# Autodesk Inventor assembly: 0070.725-R
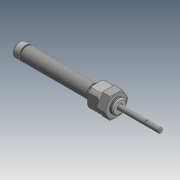
[picture p0: Inventor's stored thumbnail of the model, 180x180]
Saved by Autodesk Inventor 2020.4 (Build 244396000, 396)
## iProperties
Part Number: 0070.725-R
Catalog Web Link: www.cadenas.de
Description: Original Line Standard Air Cylinders-Standard Air Cylinders
Vendor: BIMBA
Document SubType Name: Assembly
Designer: partserver
Manufacturer: BIMBA
Mass: 4.93332 g
Surface Area: 61.3507 cm^2
Volume: 4.93332 cm^3
Density: 1 g/cm^3
Category: PARTsolutions
Company: BIMBA
PSOL_IDENT_0: {$CADENAS_DATA\23d-libs\bimba\bimba_brand\bimba_imperial\bimba_full_line\original_line_cylinders\sta
PSOL_IDENT_1: ndard_air_cylinders\standard_air_cylinder_asmtab.prj},328 {VTYP=3D},{STYP=ASSTAB},{NB=0070.725-R},{L
PSOL_IDENT_2: INA=0070.725-R},{NN=Original Line Standard Air Cylinders},{DATE=19.01.2022 10:19:38},{GEOMDATE=11.11
PSOL_IDENT_3: .2021 07:31:43},{VERSION=},{LINEID=20},{WBVAR=STROKE,ACTING,MNT,DER,NR,BM,CO,OO,VO,M,EE,EEL,K,Q,Y,G,
PSOL_IDENT_4: T,HL,B,H,SER,SR,NT,W,STPT1,STPT2,STPT3,STPT4,MB,PB,PRC,TB,MN},{WBNUMERIC=STROKE,EEL}  {NB=0070.725-R
PSOL_IDENT_5: },{LINA=0070.725-R},{KT=DUMMY},{PN=0070.725-R},{PNC=0070.725-R},{PNA=(NO ACCESSORIES)},{PNAHELP=},{D
PSOL_IDENT_6: ASH=-},{BORE1=0.31250000},{BORE=5/16\" (007)},{BOREPN=007},{STROKE=0.725},{STROKEALG=[0.011:50/0.001
PSOL_IDENT_7: ]},{STROKE1=0.725},{ACTING=R},{ACTINGALG= '' , 'Single Acting' , 'R' , 'Reverse Single Acting (R)' ,
PSOL_IDENT_8: 'D' , 'Double Acting (D)' },{ACTINGPN=R},{MNT=},{MNTALG= '' , 'Front Nose Mounting' , 'P' , 'Rear P
PSOL_IDENT_9: ivot Mounting (P)' },{TYPE=},{MNTPN=},{DER=},{DERALG= '' , 'N/A' },{NR=},{NRALG= '' , 'N/A' },{NRPN=
PSOL_IDENT_10: },{BM=},{BMALG= '' , 'N/A' },{BMPN=},{CO=},{COALG= '' , 'N/A' },{OO=},{OOALG= '', 'N/A' },{OOPN=},{V
PSOL_IDENT_11: O=Z},{VOALG= 'Z' , 'N/A' },{VOPN=},{OOVOPN=},{M=},{MALG= '', 'Without Magnet', 'M', 'With Magnet' },
PSOL_IDENT_12: {EE=},{EEL=0.000},{EEMAX=49.2750},{EEALG= '', 'Without Extra Extension', 'EE', 'With Extra Extension'
PSOL_IDENT_13: },{EELALG=0},{EEPN=},{EEPN1=0.000},{K=},{KALG= '' , 'N/A' },{KPN=},{Q=},{QALG= '' , 'N/A' },{QPN=},
PSOL_IDENT_14: {Y=},{YALG= '' , 'N/A' },{YPN=},{YCON=},{F=},{FALG= '', 'Non-Coated (Standard)', 'F', 'Molycoated' }
PSOL_IDENT_15: ,{FPN=},{G=},{GPN=},{GPN99=},{T=},{TALG= '' , 'Standard -20° to 200°F (-29° to 95°C)' , 'N' , 'Low T
PSOL_IDENT_16: emperature' , 'V' , 'High Temperature' },{NPN=},{VPN=},{HL=},{HLALG= '' , 'N/A' },{B=},{BALG= '' , '
PSOL_IDENT_17: Standard Bumpers' },{BPN=},{H=},{HALG= '', 'N/A' },{HPN=},{SER=},{SERALG= '' , 'N/A' },{SR=},{SRALG=
PSOL_IDENT_18: '' , 'Standard Stainless Steel' },{SRPN=},{SRCON=0},{NT=},{NTPN=},{W=},{WALG= '' , 'Without Wiper'
PSOL_IDENT_19: , 'W' , 'With Wiper' },{WPN=},{E=},{EALG= '' , 'Standard Seals/Lube' , 'E' , 'Non-Lube Seals/Lube' }
PSOL_IDENT_20: ,{EPN=},{ST=},{STALG= '' , 'N/A' },{STPT1=},{STPT1ALG= '' , 'N/A' },{STPT2=},{STPT2ALG= '' , 'N/A' }
PSOL_IDENT_21: ,{STPT3=},{STPT3ALG= '' , 'N/A' },{STPT4=},{STPT4ALG= '' , 'N/A' },{STPN=},{MB=},{MBALG= '' , 'Witho
PSOL_IDENT_22: ut Mounting Bracket' , 'F,D-26765' , 'D-26765 (front)' },{MBPN=},{MBPNALL=D-26765},{MBPNALLREAR=},{P
PSOL_IDENT_23: B=},{PBALG= '' , 'N/A' },{PBPN=},{PBPNALL=},{PRC=},{PRCALG= '' , 'W/out Pivot Rod Clevis' , 'F,D-266
PSOL_IDENT_24: 90' , 'D-26690 (front)' },{PRCPN=},{PRCPNALL=D-26690},{TB=},{TBALG= '' , 'N/A' },{TBPN=},{TBPNALL=},
PSOL_IDENT_25: {MN=},{MNALG= '' , 'N/A' },{MNPN=},{MNCONF=},{MNCONR=},{TLEN=1.8150},{FRAC=3.4400},{RGCON=},{RGDACCO
PSOL_IDENT_26: N=R},{RHCON=},{RHCON1=},{RHCONON=1},{RHACCON=R},{FNUTCON=1},{RNUTCON=0},{FNUTPN=D-801},{RNUTPN=},{FN
PSOL_IDENT_27: UTTRANS=0.0000},{RNUTTRANS=0.0000},{VHOLECON=0},{A1=0.8450},{A1N=0.6250},{A1P=0.8450},{A1B=0.9060},{
PSOL_IDENT_28: A4=0.1585},{A4N=0.2550},{A4P=0.1585},{A5=0.0220},{A1H=0.328},{A1NH=0.3280},{A1PH=0.8750},{A1BH=0.000
PSOL_IDENT_29: 0},{A1SH=0.0000},{A2H=0.1585},{A2NH=0.1585},{LENGTH=1.4900},{LENGTH1=1.4900},{LENGTH2=1.6500},{MUL=1
PSOL_IDENT_30: .8125},{MUL11=1.8125},{MUL22=1.8125},{MUL33=1.0875},{MUL2=1.2500},{MUL211=1.2500},{MUL222=1.2500},{M
PSOL_IDENT_31: UL233=0.7500},{SSS=1.4500},{RGLEN=0.7085},{RHLEN=0.1915},{SSS1=2.0000},{A13=0.7190},{DIF=0.0000},{G5=
PSOL_IDENT_32: 0.0000},{ON=0},{SSADD=0.0000},{BADD=0.0000},{MADD=0.0000},{NVADD=0.0000},{TRACKL=1.5090},{TRACKCON=D
PSOL_IDENT_33: -74168},{TRIMCON=0},{TRIMCON1=0},{PINCON=},{FSPACE=0.3782},{SPACE=0.0211},{TEXT=0.0369},{S1=0.5000},
PSOL_IDENT_34: {D1=0.0000},{D1N=0.3590},{D1B=0.6050},{D1P=0.0000},{FA=0.560},{RA=0.5600},{PPATH=standard_air_cylind
PSOL_IDENT_35: er_asmtpl.prj},{MATALGHTML=<b>Standard Original Line:</b><dl><dt>Rod:</dt><dd>- Stainless Steel</dd>
PSOL_IDENT_36: <dd>&nbsp;&nbsp;(5/16 9/16 Bores)</dd><dd>- High Strength Carbon Steel</dd><dd>&nbsp;&nbsp;(3/4 3 Bo
PSOL_IDENT_37: re)</dd><dd>- Stainless Steel</dd><dd>&nbsp;&nbsp;(X style DXP/DX/DXDE)</dd><dt>Bearings:</dt><dd>-
PSOL_IDENT_38: Sintered Bronze</dd><dt>Body:</dt><dd>- 304 Stainless Steel</dd><dt>End Caps:</dt><dd>- Aluminum</dd
PSOL_IDENT_39: ><dt>Seals:</dt><dd>- Buna N</dd></dl>},{ASSCFGPRA=007R},{MBPNA=},{MNPNA=},{PRCPNA=},{ASSOPTACC=STPT
PSOL_IDENT_40: 4},{A=3.44},{HADD=0.0000},{WFL=0},{QADD=0.000},{QADD1=0.200},{TEST=0.0000},{MNTB=},{STDNUTF=1},{STDN
PSOL_IDENT_41: UTR=0},{STRK2D=0},{X2D=2},{STROKESW=0.725},{EESW=0.000},{FCD=0},{BCD=0},{RCD=0},{CUSTADD=0.000},{FT=
PSOL_IDENT_42: #5-40},{FT1=#5-40},{FT2=1/2-28 UNF-2A},{PORT=#10-32},{FT11=1/2-28 UNF-2A},{FT12=3/8-24 UNF-2A},{B1=}
NB: 0070.725-R
NN: Original Line Standard Air Cylinders
NT: Threaded (Standard)
NBSYN: $PNC.
LINA: 0070.725-R
CATALOG: Bimba Products
PN: 0070.725-R
PNA: (NO ACCESSORIES)
BORE: 5/16" (007)
STROKE: 0.725
ACTING: Reverse Single Acting (R)
MNT: Front Nose
DER: N/A
NR: N/A
BM: N/A
CO: N/A
OO: N/A
VO: N/A
M: Without Magnet
EE: Without Extra Extension
EEL: 0
K: N/A
Q: N/A
Y: N/A
G: Standard Lube
T: Standard -20° to 200°F (-29° to 95°C)
HL: N/A
B: Standard Bumpers
H: N/A
SER: N/A
SR: Standard Stainless Steel
W: Without Wiper
STPT1: N/A
STPT2: N/A
STPT3: N/A
STPT4: N/A
MB: Without Mounting Bracket
PB: N/A
PRC: W/out Pivot Rod Clevis
TB: N/A
MN: N/A
A: 3.44
SUPPLIER: BIMBA
ARTICLENO: 0070.725-R
BOMINFO: 0070.725-R
CREATOR: CADENAS GmbH
Title: 0070.725-R
Author: Cadenas PARTsolutions
Comments: Standard Air Cylinders
## Documents named in this file (7)
- C:\_WORKSPACE\DATA\COMMON\BIMBA\0070_725-R.iam
- C:\_WORKSPACE\DATA\COMMON\BIMBA\0070_725-R0000000_0_dummy.ipt
- C:\_WORKSPACE\DATA\COMMON\BIMBA\007R000-0_725_rod_guide.ipt
- C:\_WORKSPACE\DATA\COMMON\BIMBA\007R-1_8150.ipt
- C:\_WORKSPACE\DATA\COMMON\BIMBA\0070000_rear_head.ipt
- C:\_WORKSPACE\DATA\COMMON\BIMBA\D-801.ipt
- C:\_WORKSPACE\DATA\COMMON\BIMBA\0070_725-R0000_rod.ipt
## Components (6 placed, 6 different names)
1. 0070_725-R0000000_0_dummy:1
2. 007R000-0_725_rod_guide:1 — Mate:1, Mate:2
3. 007R-1_8150:1
4. 0070000_rear_head:1
5. D-801:1
6. 0070_725-R0000_rod:1 — Mate:1, Mate:2
## Relationships (2: Mate 2)
- Mate:1: 007R000-0_725_rod_guide:1 ↔ 0070_725-R0000_rod:1
- Mate:2: 007R000-0_725_rod_guide:1 ↔ 0070_725-R0000_rod:1
